# Autodesk Inventor assembly: CRA-ASM-1001
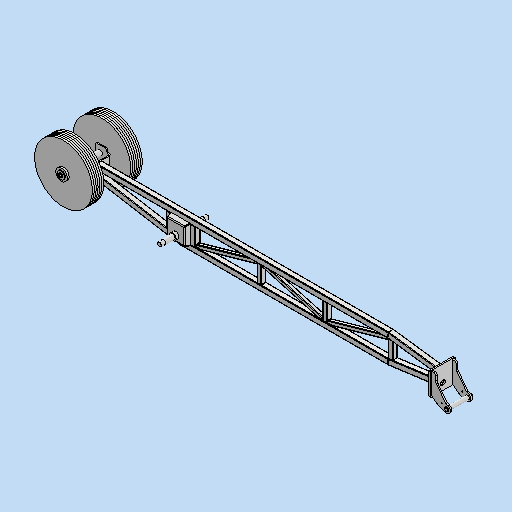
[picture p0: Inventor's stored thumbnail of the model, 512x512]
Saved by Autodesk Inventor 2025.3 (Build 293356030, 356C)
## iProperties
Created: 2025-12-20
Part Number: CRA-ASM-1001
Document SubType Name: Assembly
Designer: josh
Description: CLEANING ROBOT ARM ASSEMBLY
Author: josh
## Documents named in this file (8)
- R:\A1- Neuweg Design Data\OM Robotics\CLEANING ROBOT TOWER PROJECT\CRA-ASM-1001.iam
- R:\A1- Neuweg Design Data\OM Robotics\CLEANING ROBOT TOWER PROJECT\CRA-ASM-1002.iam
- R:\A1- Neuweg Design Data\OM Robotics\CLEANING ROBOT TOWER PROJECT\CRA-1027.ipt
- R:\A1- Neuweg Design Data\OM Robotics\CLEANING ROBOT TOWER PROJECT\CRA-1028.ipt
- R:\A1- Neuweg Design Data\OM Robotics\CLEANING ROBOT TOWER PROJECT\CRA-1029.ipt
- R:\A1- Neuweg Design Data\OM Robotics\CLEANING ROBOT TOWER PROJECT\92979A467.ipt
- R:\A1- Neuweg Design Data\OM Robotics\CLEANING ROBOT TOWER PROJECT\CRA-ASM-1003.iam
- R:\A1- Neuweg Design Data\OM Robotics\CLEANING ROBOT TOWER PROJECT\CRA-1022.ipt
## Components (22 placed, 7 different names)
1. CRA-ASM-1002:1 [sub-assembly] — Insert:1, Insert:9, Insert:19, Insert:20
2. CRA-ASM-1003:1 [sub-assembly]
3. CRA-1027:1 — Insert:1, Insert:2
4. CRA-1027:9 — Insert:5, Insert:10
5. CRA-1027:2 — Insert:2, Insert:3
6. CRA-1027:3 — Insert:3, Insert:4
7. CRA-1027:4 — Insert:4, Insert:5
8. CRA-1027:10 — Insert:10, Insert:11
9. CRA-1027:5 — Insert:14
10. CRA-1027:6
11. CRA-1027:7
12. CRA-1027:8 — Insert:9
13. CRA-1028:3 — Insert:11, Insert:15
14. CRA-1028:4 — Insert:16
15. CRA-1027:12
16. CRA-1027:11 — Insert:14
17. CRA-1029:1 — Insert:15, Insert:18
18. CRA-1029:2 — Insert:16, Insert:17
19. 92979A467:1 — Insert:17
20. 92979A467:2 — Insert:18
21. CRA-1022:1 — Insert:19
22. CRA-1022:2 — Insert:20
## Relationships (20: Insert 20)
- Insert:1: CRA-ASM-1002:1 ↔ CRA-1027:1
- Insert:2: CRA-1027:1 ↔ CRA-1027:2
- Insert:3: CRA-1027:2 ↔ CRA-1027:3
- Insert:4: CRA-1027:3 ↔ CRA-1027:4
- Insert:5: CRA-1027:9 ↔ CRA-1027:4
- [Insert]: CRA-1027:5 ↔ CRA-1027:6
- [Insert]: CRA-1027:6 ↔ CRA-1027:7
- [Insert]: CRA-1027:7 ↔ CRA-1027:8
- Insert:9: CRA-ASM-1002:1 ↔ CRA-1027:8
- Insert:10: CRA-1027:9 ↔ CRA-1027:10
- Insert:11: CRA-1027:10 ↔ CRA-1028:3
- [Insert]: CRA-1028:4 ↔ CRA-1027:12
- [Insert]: CRA-1027:12 ↔ CRA-1027:11
- Insert:14: CRA-1027:5 ↔ CRA-1027:11
- Insert:15: CRA-1028:3 ↔ CRA-1029:1
- Insert:16: CRA-1028:4 ↔ CRA-1029:2
- Insert:17: CRA-1029:2 ↔ 92979A467:1
- Insert:18: CRA-1029:1 ↔ 92979A467:2
- Insert:19: CRA-ASM-1002:1 ↔ CRA-1022:1
- Insert:20: CRA-ASM-1002:1 ↔ CRA-1022:2
## Named parameters: d5_d1 = 0 mm, d6_d2 = 0 mm, d7_d3 = 0 mm, d11_d9 = 0 mm, d12_d10 = 0 mm
